# Autodesk Inventor assembly: linac_lower_ax_mount-asm
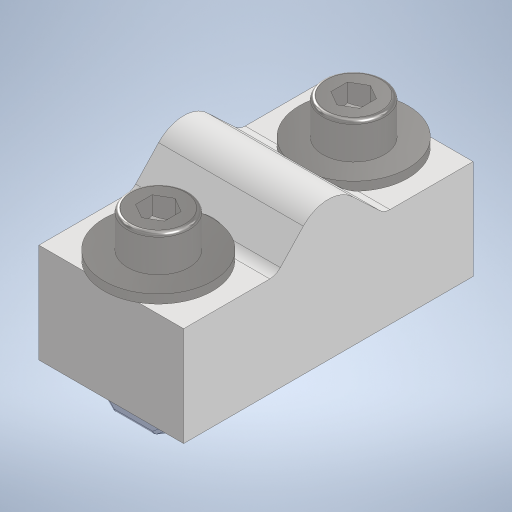
[picture p0: Inventor's stored thumbnail of the model, 512x512]
Saved by Autodesk Inventor 2024 (Build 280153000, 153)
## iProperties
Created: 2025-12-25
Part Number: linac_lower_ax_mount-asm
Document SubType Name: Assembly
Designer: schar
Author: schar
## Documents named in this file (5)
- C:\Users\schar\Desktop\projectBlueprint\AMSTS\hardware\linac_lower_ax_mount-asm.iam
- C:\Users\schar\Desktop\projectBlueprint\AMSTS\hardware\linac_lower_ax_mount.ipt
- C:\Users\schar\Documents\Inventor\Content Center Files\R2024\en-US\DIN 9021\DIN 9021 - 5,3.ipt
- C:\Users\schar\Desktop\projectBlueprint\AMSTS\hardware\tnut_m5_2020.ipt
- C:\Users\schar\Documents\Inventor\Content Center Files\R2024\en-US\ISO 4762(1)\DIN EN ISO 4762 - M5 x 20.ipt
## Components (7 placed, 4 different names)
1. linac_lower_ax_mount:1 — Mate:1, Mate:2, Mate:3, Mate:4, Rigid:1, Rigid:2, Mate:7, Mate:8
2. DIN 9021 5,3:1 — Mate:1, Mate:3, Mate:5
3. DIN 9021 5,3:2 — Mate:2, Mate:4, Mate:6
4. tnut_m5_2020:1 — Rigid:1
5. tnut_m5_2020:2 — Rigid:2
6. DIN EN ISO 4762 M5 x 20:1 — Mate:6, Mate:7
7. DIN EN ISO 4762 M5 x 20:2 — Mate:5, Mate:8
## Relationships (10: Mate 8, WeldJoint 2)
- Mate:1: linac_lower_ax_mount:1 ↔ DIN 9021 5,3:1
- Mate:2: linac_lower_ax_mount:1 ↔ DIN 9021 5,3:2
- Mate:3: linac_lower_ax_mount:1 ↔ DIN 9021 5,3:1
- Mate:4: linac_lower_ax_mount:1 ↔ DIN 9021 5,3:2
- Rigid:1 [WeldJoint] (-0.159 mm): linac_lower_ax_mount:1 ↔ tnut_m5_2020:1
- Rigid:2 [WeldJoint] (-0.159 mm): linac_lower_ax_mount:1 ↔ tnut_m5_2020:2
- Mate:5: DIN 9021 5,3:1 ↔ DIN EN ISO 4762 M5 x 20:2
- Mate:6: DIN 9021 5,3:2 ↔ DIN EN ISO 4762 M5 x 20:1
- Mate:7: linac_lower_ax_mount:1 ↔ DIN EN ISO 4762 M5 x 20:1
- Mate:8: linac_lower_ax_mount:1 ↔ DIN EN ISO 4762 M5 x 20:2
